# Autodesk Inventor assembly: MIRleftMIRright脚一枚
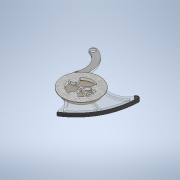
[picture p0: Inventor's stored thumbnail of the model, 180x180]
Saved by Autodesk Inventor 2020.2 (Build 242310000, 310)
## iProperties
Created: 2020-04-13
Part Number: MIRleftMIRright脚一枚
Document SubType Name: Assembly
Designer: aoyama
Mass: 31.6013 g
Surface Area: 259.988 cm^2
Volume: 17.8864 cm^3
Density: 1.76678 g/cm^3
Author: aoyama
## Documents named in this file (8)
- C:\Users\aoyam\Desktop\SRDC_local\Inventor\二年機\インナー4層丙参型\脚\ネジクランク\MIR達\MIRleftMIRright脚一枚.iam
- C:\Users\aoyam\Desktop\SRDC_local\Inventor\二年機\インナー4層丙参型\脚\ネジクランク\MIR達\MIRleftMIRrightクランク3t.ipt
- C:\Users\aoyam\Desktop\SRDC_local\Inventor\二年機\インナー4層丙参型\脚\ネジクランク\MIR達\MIRleftMIRrightクランク4t.ipt
- C:\Users\aoyam\Desktop\SRDC_local\Inventor\二年機\インナー4層丙参型\汎用部品\MIR達\MIRleftMIRrightベアリングd3D8B4F無.ipt
- C:\Users\aoyam\Desktop\SRDC_local\Inventor\二年機\インナー4層丙参型\脚\ネジクランク\MIR達\MIRleftMIRrightヘッケン改.ipt
- C:\Users\aoyam\Desktop\SRDC_local\Inventor\二年機\インナー4層丙参型\脚\ネジクランク\MIR達\MIRleftMIRright揺動節.ipt
- C:\Users\aoyam\Desktop\SRDC_local\Inventor\二年機\インナー4層丙参型\汎用部品\MIR達\MIRleftMIRrightオイレス外径8内径6L2.ipt
- C:\Users\aoyam\Desktop\SRDC_local\Inventor\二年機\インナー4層丙参型\脚\ネジクランク\MIR達\MIRleftMIRright脚ゴム.ipt
## Components (9 placed, 7 different names)
1. MIRleftMIRrightクランク3t:1 — 挿入:16, 挿入:15, 挿入:17
2. MIRleftMIRrightクランク4t:1 — 挿入:16, 挿入:14, 挿入:13, 挿入:12
3. MIRleftMIRrightベアリングd3D8B4F無:1 — 挿入:14
4. MIRleftMIRrightベアリングd3D8B4F無:2 — 挿入:13, 挿入:15
5. MIRleftMIRrightベアリングd3D8B4F無:3 — 挿入:12
6. MIRleftMIRrightヘッケン改:1 — 挿入:17, 挿入:11, 挿入:8, 挿入:9, メイト:1
7. MIRleftMIRright揺動節:1 — 挿入:11
8. MIRleftMIRrightオイレス外径8内径6L2:1 — 挿入:8
9. MIRleftMIRright脚ゴム:1 — 挿入:9, メイト:1
## Relationships (10: Insert 9, Mate 1)
- 挿入:16 [Insert]: MIRleftMIRrightクランク3t:1 ↔ MIRleftMIRrightクランク4t:1
- 挿入:14 [Insert]: MIRleftMIRrightクランク4t:1 ↔ MIRleftMIRrightベアリングd3D8B4F無:1
- 挿入:13 [Insert]: MIRleftMIRrightクランク4t:1 ↔ MIRleftMIRrightベアリングd3D8B4F無:2
- 挿入:15 [Insert]: MIRleftMIRrightクランク3t:1 ↔ MIRleftMIRrightベアリングd3D8B4F無:2
- 挿入:12 [Insert]: MIRleftMIRrightクランク4t:1 ↔ MIRleftMIRrightベアリングd3D8B4F無:3
- 挿入:17 [Insert] (0.2 mm): MIRleftMIRrightクランク3t:1 ↔ MIRleftMIRrightヘッケン改:1
- 挿入:11 [Insert]: MIRleftMIRrightヘッケン改:1 ↔ MIRleftMIRright揺動節:1
- 挿入:8 [Insert]: MIRleftMIRrightヘッケン改:1 ↔ MIRleftMIRrightオイレス外径8内径6L2:1
- 挿入:9 [Insert]: MIRleftMIRrightヘッケン改:1 ↔ MIRleftMIRright脚ゴム:1
- メイト:1 [Mate]: MIRleftMIRrightヘッケン改:1 ↔ MIRleftMIRright脚ゴム:1
